# Autodesk Inventor assembly: RV-2AJ
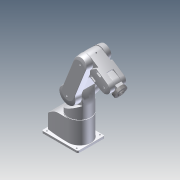
[picture p0: Inventor's stored thumbnail of the model, 180x180]
Saved by Autodesk Inventor 2015 (Build 190159000, 159)
## iProperties
Created: 2016-11-14
Part Number: RV-2AJ
Document SubType Name: Assembly
Designer: taka
Mass: 17177.4 g
Surface Area: 7181.76 cm^2
Volume: 13315.8 cm^3
Density: 1.29 g/cm^3
Author: taka
## Documents named in this file (7)
- C:\Users\taka\Documents\Inventor\5DOF\RV-2AJ.iam
- C:\Users\taka\Documents\Inventor\5DOF\インポートされたコンポーネント\Assem1\Link1.ipt
- C:\Users\taka\Documents\Inventor\5DOF\インポートされたコンポーネント\Assem1\Link2.ipt
- C:\Users\taka\Documents\Inventor\5DOF\インポートされたコンポーネント\Assem1\Link3.ipt
- C:\Users\taka\Documents\Inventor\5DOF\インポートされたコンポーネント\Assem1\Link4.ipt
- C:\Users\taka\Documents\Inventor\5DOF\インポートされたコンポーネント\Assem1\Link5.ipt
- C:\Users\taka\Documents\Inventor\5DOF\J7.ipt
## Components (6 placed, 6 different names)
1. Link1:1 — 挿入:1
2. Link2:1 — 挿入:1, 挿入:6
3. Link3:1 — 挿入:6, 挿入:7
4. Link4:1 — 挿入:7, 挿入:8
5. Link5:1 — 挿入:5, 挿入:8
6. J7:1 — 挿入:5
## Relationships (5: Insert 5)
- 挿入:1 [Insert]: Link1:1 ↔ Link2:1
- 挿入:5 [Insert]: Link5:1 ↔ J7:1
- 挿入:6 [Insert] (2 mm): Link2:1 ↔ Link3:1
- 挿入:7 [Insert] (3 mm): Link3:1 ↔ Link4:1
- 挿入:8 [Insert] (1 mm): Link4:1 ↔ Link5:1
